# Autodesk Inventor assembly: Ensamble EVA
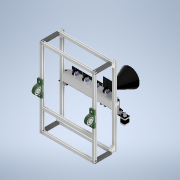
[picture p0: Inventor's stored thumbnail of the model, 180x180]
Saved by Autodesk Inventor 2020.3 (Build 243373000, 373)
## iProperties
Created: 2021-02-22
Part Number: Ensamble EVA
Document SubType Name: Assembly
Designer: juanp
Author: juanp
## Documents named in this file (13)
- C:\Users\juanp\Desktop\Robocol\Nuevo EVA\V1\Ensamble EVA.iam
- C:\Users\juanp\Desktop\Robocol\Nuevo EVA\Recursos\Actuador Lineal\Actuador Lineal (sin carro).iam
- C:\Users\juanp\Desktop\Robocol\Nuevo EVA\Recursos\Chasis\Diseño 1.3 (2020)\Ensamble_chasis.iam
- C:\Users\juanp\Desktop\Robocol\Nuevo EVA\Recursos\Actuador Lineal\Carro deslizante\Carro Deslizante.ipt
- C:\Users\juanp\Desktop\Robocol\Nuevo EVA\V1\Dispensador\Dispensador V1.iam
- C:\Users\juanp\Desktop\Robocol\Nuevo EVA\V1\Cajas\cajas.iam
- C:\Users\juanp\Desktop\Robocol\Nuevo EVA\Recursos\Actuador Lineal\Partes\VSLOT 2020 Extrusion Mini.ipt
- C:\Users\juanp\Desktop\Robocol\Nuevo EVA\Recursos\Pi Camera\RspCameraMia.iam
- C:\Users\juanp\Desktop\Robocol\Nuevo EVA\Recursos\Acople a chasis\Platinas de unión.ipt
- C:\Users\juanp\Desktop\Robocol\Nuevo EVA\Recursos\Acople a chasis\Soporte Cajas.ipt
- C:\Users\juanp\Desktop\Robocol\Nuevo EVA\Recursos\Pi Camera\Case.ipt
- C:\Users\juanp\Desktop\Robocol\Nuevo EVA\Recursos\Acople a chasis\Soporte Actuador.ipt
- C:\Users\juanp\Desktop\Robocol\Nuevo EVA\Recursos\Acople a chasis\Soporte Actuador MIR.ipt
## Components (17 placed, 12 different names)
1. Actuador Lineal (sin carro):1 [sub-assembly] — Angle:1, Angle:2, Mate:1, Angle:3, Angle:4, Flush:2, Mate:3, Flush:10, Mate:20, Mate:21, Mate:24, Mate:45, Mate:47
2. Ensamble_chasis:1 [sub-assembly] — Angle:1, Angle:2, Mate:1, Angle:5, Flush:11, Mate:19, Mate:23, Flush:13, Flush:15, Mate:31, Mate:32, Mate:33, Flush:23
3. Carro Deslizante:1 — Angle:3, Angle:4, Flush:2, Mate:3, Mate:4, Mate:5, Mate:6, Angle:6, Angle:7
4. Dispensador V1:1 [sub-assembly] — Mate:4, Mate:5, Mate:6, Mate:7, Mate:25, Mate:27, Mate:42, Mate:43
5. cajas:1 [sub-assembly] — Angle:5, Mate:7, Flush:10, Mate:25, Mate:35, Mate:36, Mate:37, Flush:24
6. VSLOT 2020 Extrusion Mini:1 — Flush:11, Mate:19, Mate:20, Mate:21, Flush:15, Flush:20, Flush:21, Flush:22, Mate:38, Mate:46, Flush:26
7. VSLOT 2020 Extrusion Mini:2 — Mate:23, Flush:13, Mate:24, Mate:30, Flush:16, Flush:17, Flush:18, Flush:19, Mate:34, Mate:44, Flush:25
8. RspCameraMia:1 [sub-assembly] — Angle:6, Mate:27, Mate:39, Mate:40, Mate:41
9. Platinas de unión:1 — Mate:30, Flush:16, Flush:17
10. Platinas de unión:2 — Mate:32, Flush:20, Flush:21
11. Platinas de unión:3 — Mate:31, Flush:18, Flush:19
12. Platinas de unión:4 — Mate:33, Flush:22, Flush:23
13. Soporte Cajas:1 — Mate:34, Mate:35, Mate:36
14. Soporte Cajas:2 — Mate:37, Flush:24, Mate:38
15. Case:1 — Mate:39, Mate:40, Mate:41, Angle:7, Mate:42, Mate:43
16. Soporte Actuador:1 — Mate:44, Flush:25, Mate:45
17. Soporte Actuador MIR:1 — Mate:46, Flush:26, Mate:47
## Relationships (54: Mate 31, Flush 16, Angle 7)
- Angle:1 (180 deg): Actuador Lineal (sin carro):1 ↔ Ensamble_chasis:1
- Angle:2 (0 deg): Actuador Lineal (sin carro):1 ↔ Ensamble_chasis:1
- Mate:1: Actuador Lineal (sin carro):1 ↔ Ensamble_chasis:1
- Angle:3 (0 deg): Actuador Lineal (sin carro):1 ↔ Carro Deslizante:1
- Angle:4 (180 deg): Actuador Lineal (sin carro):1 ↔ Carro Deslizante:1
- Flush:2: Actuador Lineal (sin carro):1 ↔ Carro Deslizante:1
- Mate:3: Actuador Lineal (sin carro):1 ↔ Carro Deslizante:1
- Mate:4: Carro Deslizante:1 ↔ Dispensador V1:1
- Mate:5: Carro Deslizante:1 ↔ Dispensador V1:1
- Mate:6: Carro Deslizante:1 ↔ Dispensador V1:1
- Angle:5 (0 deg): Ensamble_chasis:1 ↔ cajas:1
- Mate:7 (4.167 mm): Dispensador V1:1 ↔ cajas:1
- Flush:10: Actuador Lineal (sin carro):1 ↔ cajas:1
- Flush:11: Ensamble_chasis:1 ↔ VSLOT 2020 Extrusion Mini:1
- Mate:19: Ensamble_chasis:1 ↔ VSLOT 2020 Extrusion Mini:1
- Mate:20: Actuador Lineal (sin carro):1 ↔ VSLOT 2020 Extrusion Mini:1
- Mate:21: Actuador Lineal (sin carro):1 ↔ VSLOT 2020 Extrusion Mini:1
- Mate:23: Ensamble_chasis:1 ↔ VSLOT 2020 Extrusion Mini:2
- Flush:13: Ensamble_chasis:1 ↔ VSLOT 2020 Extrusion Mini:2
- Mate:24: Actuador Lineal (sin carro):1 ↔ VSLOT 2020 Extrusion Mini:2
- Flush:15 (250 mm): Ensamble_chasis:1 ↔ VSLOT 2020 Extrusion Mini:1
- Mate:25: Dispensador V1:1 ↔ cajas:1
- Angle:6 (135 deg): Carro Deslizante:1 ↔ RspCameraMia:1
- Mate:27: Dispensador V1:1 ↔ RspCameraMia:1
- Mate:30: VSLOT 2020 Extrusion Mini:2 ↔ Platinas de unión:1
- Flush:16: VSLOT 2020 Extrusion Mini:2 ↔ Platinas de unión:1
- Flush:17 (2.5 mm): VSLOT 2020 Extrusion Mini:2 ↔ Platinas de unión:1
- Mate:31: Ensamble_chasis:1 ↔ Platinas de unión:3
- Flush:18: VSLOT 2020 Extrusion Mini:2 ↔ Platinas de unión:3
- Flush:19 (2.5 mm): VSLOT 2020 Extrusion Mini:2 ↔ Platinas de unión:3
- Mate:32: Ensamble_chasis:1 ↔ Platinas de unión:2
- Flush:20 (2.5 mm): VSLOT 2020 Extrusion Mini:1 ↔ Platinas de unión:2
- Flush:21: VSLOT 2020 Extrusion Mini:1 ↔ Platinas de unión:2
- Mate:33: Ensamble_chasis:1 ↔ Platinas de unión:4
- Flush:22: VSLOT 2020 Extrusion Mini:1 ↔ Platinas de unión:4
- Flush:23 (2.5 mm): Ensamble_chasis:1 ↔ Platinas de unión:4
- Mate:34: VSLOT 2020 Extrusion Mini:2 ↔ Soporte Cajas:1
- Mate:35: cajas:1 ↔ Soporte Cajas:1
- Mate:36 (-27 mm): cajas:1 ↔ Soporte Cajas:1
- Mate:37: cajas:1 ↔ Soporte Cajas:2
- Flush:24 (-27 mm): cajas:1 ↔ Soporte Cajas:2
- Mate:38: VSLOT 2020 Extrusion Mini:1 ↔ Soporte Cajas:2
- Mate:39: RspCameraMia:1 ↔ Case:1
- Mate:40: RspCameraMia:1 ↔ Case:1
- Mate:41: RspCameraMia:1 ↔ Case:1
- Angle:7 (0 deg): Carro Deslizante:1 ↔ Case:1
- Mate:42: Dispensador V1:1 ↔ Case:1
- Mate:43: Dispensador V1:1 ↔ Case:1
- Mate:44: VSLOT 2020 Extrusion Mini:2 ↔ Soporte Actuador:1
- Flush:25: VSLOT 2020 Extrusion Mini:2 ↔ Soporte Actuador:1
- Mate:45: Actuador Lineal (sin carro):1 ↔ Soporte Actuador:1
- Mate:46: VSLOT 2020 Extrusion Mini:1 ↔ Soporte Actuador MIR:1
- Flush:26: VSLOT 2020 Extrusion Mini:1 ↔ Soporte Actuador MIR:1
- Mate:47: Actuador Lineal (sin carro):1 ↔ Soporte Actuador MIR:1
